# Autodesk Inventor assembly: slider assembly
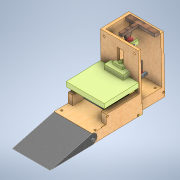
[picture p0: Inventor's stored thumbnail of the model, 180x180]
Saved by Autodesk Inventor 2021 (Build 250183000, 183)
## iProperties
Created: 2021-07-03
Part Number: slider assembly
Document SubType Name: Assembly
Designer: Rajeev
Author: Rajeev
## Documents named in this file (8)
- C:\Users\Ashwin\OneDrive\Documents\Moulding Model\vertical slider mech.iam
- C:\Users\Ashwin\OneDrive\Documents\Moulding Model\compression wheel.ipt
- C:\Users\Ashwin\OneDrive\Documents\Moulding Model\stand.ipt
- C:\Users\Ashwin\OneDrive\Documents\Moulding Model\pusher.ipt
- C:\Users\Ashwin\OneDrive\Documents\Moulding Model\Moulding final.iam
- C:\Users\Ashwin\OneDrive\Documents\Moulding Model\upper plate.ipt
- C:\Users\Ashwin\OneDrive\Documents\box.ipt
- C:\Users\Ashwin\OneDrive\Documents\part.ipt
## Components (8 placed, 7 different names)
1. Moulding final:1 [sub-assembly] — Rigid:1
2. compression wheel:2 — Mate:5, Flush:2, Mate:6, Flush:3, Angle:1
3. stand:2 — Mate:5, Flush:2, Rigid:1
4. upper plate:1 — Mate:6, Flush:3
5. box:1 — Mate:7, Flush:4
6. compression wheel:3 — Mate:7, Flush:4, Mate:8, Flush:5, Angle:2
7. pusher:1 — Mate:8, Flush:5
8. part:1
## Relationships (11: Mate 4, Flush 4, Angle 2, WeldJoint 1)
- Mate:5: compression wheel:2 ↔ stand:2
- Flush:2: compression wheel:2 ↔ stand:2
- Rigid:1 [WeldJoint]: Moulding final:1 ↔ stand:2
- Mate:6: compression wheel:2 ↔ upper plate:1
- Flush:3: compression wheel:2 ↔ upper plate:1
- Mate:7: box:1 ↔ compression wheel:3
- Flush:4: box:1 ↔ compression wheel:3
- Mate:8: compression wheel:3 ↔ pusher:1
- Flush:5: compression wheel:3 ↔ pusher:1
- Angle:1 (380 deg): compression wheel:2
- Angle:2 (24 deg): compression wheel:3
